# Autodesk Inventor assembly: arm assembly-minimodel
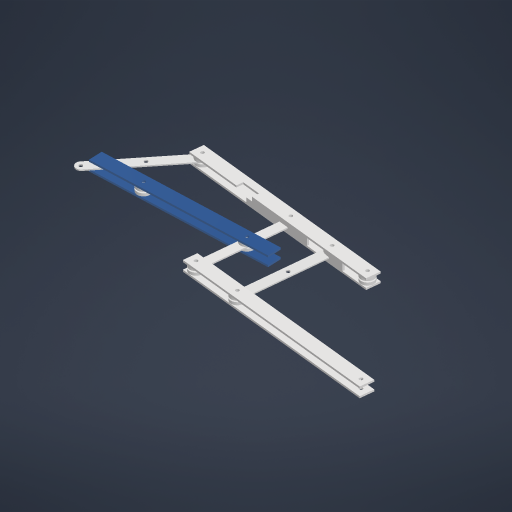
[picture p0: Inventor's stored thumbnail of the model, 512x512]
Saved by Autodesk Inventor 2024.2 (Build 282272000, 272)
## iProperties
Created: 2024-01-19
Part Number: arm assembly-minimodel
Document SubType Name: Assembly
Designer: ctam0
Author: ctam0
## Documents named in this file (6)
- C:\Users\ctam0\Downloads\TRACER DOCUMENTS 1-13-2024\Arm Completed\arm assembly-minimodel.iam
- C:\Users\ctam0\Downloads\TRACER DOCUMENTS 1-13-2024\Arm Completed\ArmPart2Mini.ipt
- C:\Users\ctam0\Downloads\TRACER DOCUMENTS 1-13-2024\Arm Completed\ArmPart3Mini.ipt
- C:\Users\ctam0\Downloads\TRACER DOCUMENTS 1-13-2024\Arm Completed\ArmPart1Mini.ipt
- C:\Users\ctam0\Downloads\TRACER DOCUMENTS 1-13-2024\Arm Completed\ArmSpacerMini.ipt
- C:\Users\ctam0\Downloads\TRACER DOCUMENTS 1-13-2024\Arm Completed\ArmConnector1Mini.ipt
## Components (22 placed, 5 different names)
1. ArmPart2Mini:1 — Angle:1, Mate:13, Mate:14, Mate:15, Mate:16, Angle:2, Angle:3, Angle:4
2. ArmPart3Mini:1 — Mate:2, Mate:3, Angle:1, Angle:2, Mate:20, Angle:3, Mate:26, Mate:30, Mate:31
3. ArmPart1Mini:1 — Angle:4, Mate:32, Mate:33, Mate:34, Mate:35, Mate:36, Mate:38, Mate:39, Mate:41, Mate:42, Mate:43, Mate:44, Mate:45, Mate:46, Mate:47, Mate:48, Mate:49, Mate:50
4. ArmSpacerMini:1 — Mate:33, Mate:41
5. ArmSpacerMini:2 — Mate:32, Mate:42
6. ArmSpacerMini:3 — Mate:3, Mate:30
7. ArmSpacerMini:4 — Mate:20, Mate:29, Mate:31
8. ArmSpacerMini:5 — Mate:34, Mate:43, Mate:48, Mate:51
9. ArmSpacerMini:6 — Mate:36, Mate:47, Mate:52
10. ArmSpacerMini:7 — Mate:35, Mate:44
11. ArmSpacerMini:8 — Mate:38, Mate:45
12. ArmSpacerMini:9 — Mate:49, Mate:50
13. ArmSpacerMini:10 — Mate:39, Mate:46, Mate:53
14. ArmSpacerMini:11 — Mate:14, Mate:18, Mate:19
15. ArmSpacerMini:12 — Mate:13, Mate:17
16. ArmSpacerMini:13 — Mate:16
17. ArmSpacerMini:14 — Mate:15
18. ArmSpacerMini:15 — Mate:2, Insert:1
19. ArmSpacerMini:16 — Mate:26, Mate:27
20. ArmConnector1Mini:1 — Mate:29, Mate:51
21. ArmConnector1Mini:2 — Mate:18, Mate:19, Mate:17, Insert:1, Mate:27, Mate:52
22. ArmConnector1Mini:3 — Mate:53
## Relationships (40: Mate 35, Angle 4, Insert 1)
- Mate:2: ArmPart3Mini:1 ↔ ArmSpacerMini:15
- Mate:3: ArmPart3Mini:1 ↔ ArmSpacerMini:3
- Angle:1 (0 deg): ArmPart2Mini:1 ↔ ArmPart3Mini:1
- Mate:13: ArmPart2Mini:1 ↔ ArmSpacerMini:12
- Mate:14: ArmPart2Mini:1 ↔ ArmSpacerMini:11
- Mate:15: ArmPart2Mini:1 ↔ ArmSpacerMini:14
- Mate:16: ArmPart2Mini:1 ↔ ArmSpacerMini:13
- Angle:2 (90 deg): ArmPart2Mini:1 ↔ ArmPart3Mini:1
- Mate:18: ArmSpacerMini:11 ↔ ArmConnector1Mini:2
- Mate:19: ArmSpacerMini:11 ↔ ArmConnector1Mini:2
- Mate:17: ArmSpacerMini:12 ↔ ArmConnector1Mini:2
- Mate:20: ArmPart3Mini:1 ↔ ArmSpacerMini:4
- Angle:3 (0 deg): ArmPart2Mini:1 ↔ ArmPart3Mini:1
- Insert:1: ArmSpacerMini:15 ↔ ArmConnector1Mini:2
- Mate:26: ArmPart3Mini:1 ↔ ArmSpacerMini:16
- Mate:27: ArmSpacerMini:16 ↔ ArmConnector1Mini:2
- Mate:29: ArmSpacerMini:4 ↔ ArmConnector1Mini:1
- Mate:30: ArmPart3Mini:1 ↔ ArmSpacerMini:3
- Mate:31: ArmPart3Mini:1 ↔ ArmSpacerMini:4
- Angle:4 (0 deg): ArmPart2Mini:1 ↔ ArmPart1Mini:1
- Mate:32: ArmPart1Mini:1 ↔ ArmSpacerMini:2
- Mate:33: ArmPart1Mini:1 ↔ ArmSpacerMini:1
- Mate:34: ArmPart1Mini:1 ↔ ArmSpacerMini:5
- Mate:35: ArmPart1Mini:1 ↔ ArmSpacerMini:7
- Mate:36: ArmPart1Mini:1 ↔ ArmSpacerMini:6
- Mate:38: ArmPart1Mini:1 ↔ ArmSpacerMini:8
- Mate:39: ArmPart1Mini:1 ↔ ArmSpacerMini:10
- Mate:41: ArmPart1Mini:1 ↔ ArmSpacerMini:1
- Mate:42: ArmPart1Mini:1 ↔ ArmSpacerMini:2
- Mate:43: ArmPart1Mini:1 ↔ ArmSpacerMini:5
- Mate:44: ArmPart1Mini:1 ↔ ArmSpacerMini:7
- Mate:45: ArmPart1Mini:1 ↔ ArmSpacerMini:8
- Mate:46: ArmPart1Mini:1 ↔ ArmSpacerMini:10
- Mate:47: ArmPart1Mini:1 ↔ ArmSpacerMini:6
- Mate:48: ArmPart1Mini:1 ↔ ArmSpacerMini:5
- Mate:49: ArmPart1Mini:1 ↔ ArmSpacerMini:9
- Mate:50: ArmPart1Mini:1 ↔ ArmSpacerMini:9
- Mate:51: ArmSpacerMini:5 ↔ ArmConnector1Mini:1
- Mate:52: ArmSpacerMini:6 ↔ ArmConnector1Mini:2
- Mate:53: ArmSpacerMini:10 ↔ ArmConnector1Mini:3
